# Autodesk Inventor assembly: Assembly5
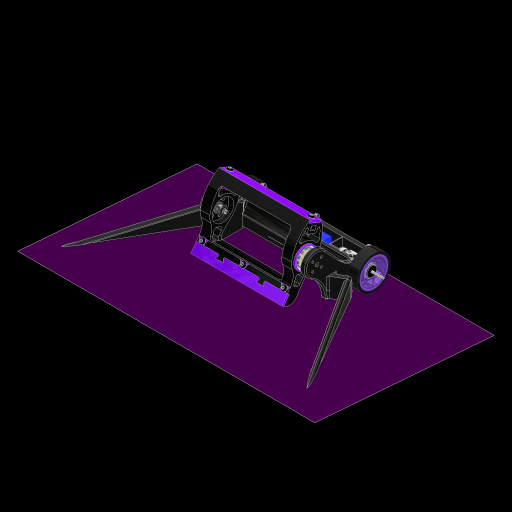
[picture p0: Inventor's stored thumbnail of the model, 512x512]
Saved by Autodesk Inventor 2024.2 (Build 282272000, 272)
## iProperties
Created: 2023-02-15
Part Number: Assembly5
Document SubType Name: Assembly
Designer: tandu
Mass: 460.972 g
Surface Area: 1632.87 cm^2
Volume: 253.693 cm^3
Density: 1.81704 g/cm^3
Author: tandu
## Documents named in this file (16)
- C:\Users\tandu\Documents\GitHub\GrabCAD\Insomnia 2020\Versions\10 Shuffler\WheeledVersion\Assembly5.iam
- C:\Users\tandu\Documents\GitHub\GrabCAD\Insomnia 2020\Versions\10 Shuffler\WheeledVersion\ChassisWheeled.ipt
- C:\Users\tandu\Documents\GitHub\GrabCAD\Insomnia 2020\Versions\10 Shuffler\WheeledVersion\Weapon\DrumAssembly.iam
- C:\Users\tandu\Documents\GitHub\GrabCAD\Insomnia 2020\Versions\10 Shuffler\WheeledVersion\BatteryMockup.ipt
- C:\Users\tandu\Documents\GitHub\GrabCAD\Insomnia 2020\Versions\10 Shuffler\WheeledVersion\Repeat Drive Mini Mk2.iam
- C:\Users\tandu\Documents\GitHub\GrabCAD\Insomnia 2020\Versions\10 Shuffler\WheeledVersion\2207 5 fixed motor.ipt
- C:\Users\tandu\Documents\GitHub\GrabCAD\Insomnia 2020\Versions\10 Shuffler\WheeledVersion\CorrectSizeWheelsIThink.ipt
- C:\Users\tandu\Documents\GitHub\GrabCAD\Insomnia 2020\Versions\10 Shuffler\WheeledVersion\WedgeTPUPiece.ipt
- C:\Users\tandu\Documents\GitHub\GrabCAD\Insomnia 2020\Versions\10 Shuffler\WheeledVersion\WedgeTPUPiece_MIR.ipt
- C:\Users\tandu\Documents\GitHub\GrabCAD\Insomnia 2020\Versions\10 Shuffler\WheeledVersion\90417A126_Phillips Rounded Head Thread-Forming Screws.ipt
- C:\Users\tandu\Documents\GitHub\GrabCAD\Insomnia 2020\Versions\10 Shuffler\WheeledVersion\57155K571_Flanged Ball Bearing.ipt
- C:\Users\tandu\Documents\GitHub\GrabCAD\Insomnia 2020\Versions\10 Shuffler\WheeledVersion\94361A593_Short-Thread Alloy Steel Shoulder Screw.ipt
- C:\Users\tandu\Documents\GitHub\GrabCAD\Insomnia 2020\Versions\10 Shuffler\WheeledVersion\Weapon\90237A110_High-Strength Steel Nylon-Insert Locknuts.ipt
- C:\Users\tandu\Documents\GitHub\GrabCAD\Insomnia 2020\Versions\10 Shuffler\WheeledVersion\DerivedLid.ipt
- C:\Users\tandu\Documents\GitHub\GrabCAD\Insomnia 2020\Versions\13 Anti Horizontal\NewWheels\Wide Wheel\WideWheelCore.ipt
- C:\Users\tandu\Documents\GitHub\GrabCAD\Insomnia 2020\Versions\13 Anti Horizontal\NewWheels\banebots 3mm hub.iam
## Components (29 placed, 15 different names)
1. ChassisWheeled:1 — Insert:1, Insert:2, Mate:1, Mate:2, Insert:3, Insert:4, Insert:6, Insert:7, Mate:3, Mate:4, Insert:8, Insert:9, Insert:10, Insert:11, Insert:13, Insert:14, Insert:15, Insert:16, Insert:19, Insert:21, Insert:22, Insert:29, Insert:30
2. BatteryMockup:1 — Mate:1, Mate:2
3. Repeat Drive Mini Mk2:1 [sub-assembly] — Insert:1
4. Repeat Drive Mini Mk2:2 [sub-assembly] — Insert:2
5. CorrectSizeWheelsIThink:1 — Insert:6
6. CorrectSizeWheelsIThink:2 — Insert:7, Tangent:1
7. WedgeTPUPiece:1 — Mate:3, Insert:8, Insert:9, Mate:5
8. WedgePiece_MIR:1 — Mate:4, Insert:10, Insert:11, Mate:6
9. DerivedLid:1 — Insert:21, Insert:22, Insert:23, Insert:24, Insert:25, Insert:26, Insert:27, Insert:28
10. WideWheelCore:1 — Insert:32, Mate:9
11. WideWheelCore:2 — Insert:31, Mate:8
12. banebots 3mm hub:1 [sub-assembly] — Insert:29, Insert:32, Mate:9
13. banebots 3mm hub:2 [sub-assembly] — Insert:30, Insert:31, Mate:8
14. 90417A126_Phillips Rounded Head Thread-Forming Screws:5 — Insert:23
15. 90417A126_Phillips Rounded Head Thread-Forming Screws:6 — Insert:25
16. 90417A126_Phillips Rounded Head Thread-Forming Screws:7 — Insert:28
17. 90417A126_Phillips Rounded Head Thread-Forming Screws:8 — Insert:24
18. 90417A126_Phillips Rounded Head Thread-Forming Screws:9 — Insert:26
19. 90417A126_Phillips Rounded Head Thread-Forming Screws:10 — Insert:27
20. 90417A126_Phillips Rounded Head Thread-Forming Screws:1 — Insert:14
21. 90417A126_Phillips Rounded Head Thread-Forming Screws:2 — Insert:15
22. 90417A126_Phillips Rounded Head Thread-Forming Screws:3 — Insert:13
23. 90417A126_Phillips Rounded Head Thread-Forming Screws:4 — Insert:16
24. DrumAssembly:1 [sub-assembly] — Insert:5, Insert:17, Insert:18
25. 2207 5 fixed motor:1 — Insert:3, Insert:4, Insert:5
26. 57155K571_Flanged Ball Bearing:2 — Insert:17
27. 57155K571_Flanged Ball Bearing:3 — Insert:18, Insert:20
28. 94361A593_Short-Thread Alloy Steel Shoulder Screw:1 — Insert:19
29. 90237A110_High-Strength Steel Nylon-Insert Locknuts:1 — Insert:20
## Relationships (41: Insert 31, Mate 9, Tangent 1)
- Insert:1: ChassisWheeled:1 ↔ Repeat Drive Mini Mk2:1
- Insert:2: ChassisWheeled:1 ↔ Repeat Drive Mini Mk2:2
- Mate:1: ChassisWheeled:1 ↔ BatteryMockup:1
- Mate:2: ChassisWheeled:1 ↔ BatteryMockup:1
- Insert:3: ChassisWheeled:1 ↔ 2207 5 fixed motor:1
- Insert:4: ChassisWheeled:1 ↔ 2207 5 fixed motor:1
- Insert:5: DrumAssembly:1 ↔ 2207 5 fixed motor:1
- Insert:6: ChassisWheeled:1 ↔ CorrectSizeWheelsIThink:1
- Insert:7: ChassisWheeled:1 ↔ CorrectSizeWheelsIThink:2
- Mate:3: ChassisWheeled:1 ↔ WedgeTPUPiece:1
- Mate:4: ChassisWheeled:1 ↔ WedgePiece_MIR:1
- Insert:8: ChassisWheeled:1 ↔ WedgeTPUPiece:1
- Insert:9: ChassisWheeled:1 ↔ WedgeTPUPiece:1
- Insert:10: ChassisWheeled:1 ↔ WedgePiece_MIR:1
- Insert:11: ChassisWheeled:1 ↔ WedgePiece_MIR:1
- Insert:13: ChassisWheeled:1 ↔ 90417A126_Phillips Rounded Head Thread-Forming Screws:3
- Insert:14: ChassisWheeled:1 ↔ 90417A126_Phillips Rounded Head Thread-Forming Screws:1
- Insert:15: ChassisWheeled:1 ↔ 90417A126_Phillips Rounded Head Thread-Forming Screws:2
- Insert:16: ChassisWheeled:1 ↔ 90417A126_Phillips Rounded Head Thread-Forming Screws:4
- Insert:17: DrumAssembly:1 ↔ 57155K571_Flanged Ball Bearing:2
- Insert:18: DrumAssembly:1 ↔ 57155K571_Flanged Ball Bearing:3
- Insert:19: ChassisWheeled:1 ↔ 94361A593_Short-Thread Alloy Steel Shoulder Screw:1
- Insert:20: 57155K571_Flanged Ball Bearing:3 ↔ 90237A110_High-Strength Steel Nylon-Insert Locknuts:1
- Mate:5: WedgeTPUPiece:1
- Mate:6: WedgePiece_MIR:1
- Mate:7
- Tangent:1: CorrectSizeWheelsIThink:2
- Insert:21: ChassisWheeled:1 ↔ DerivedLid:1
- Insert:22: ChassisWheeled:1 ↔ DerivedLid:1
- Insert:23: DerivedLid:1 ↔ 90417A126_Phillips Rounded Head Thread-Forming Screws:5
- Insert:24: DerivedLid:1 ↔ 90417A126_Phillips Rounded Head Thread-Forming Screws:8
- Insert:25: DerivedLid:1 ↔ 90417A126_Phillips Rounded Head Thread-Forming Screws:6
- Insert:26: DerivedLid:1 ↔ 90417A126_Phillips Rounded Head Thread-Forming Screws:9
- Insert:27: DerivedLid:1 ↔ 90417A126_Phillips Rounded Head Thread-Forming Screws:10
- Insert:28: DerivedLid:1 ↔ 90417A126_Phillips Rounded Head Thread-Forming Screws:7
- Insert:29: ChassisWheeled:1 ↔ banebots 3mm hub:1
- Insert:30: ChassisWheeled:1 ↔ banebots 3mm hub:2
- Insert:31: WideWheelCore:2 ↔ banebots 3mm hub:2
- Mate:8: WideWheelCore:2 ↔ banebots 3mm hub:2
- Insert:32: WideWheelCore:1 ↔ banebots 3mm hub:1
- Mate:9: WideWheelCore:1 ↔ banebots 3mm hub:1
